# Autodesk Inventor assembly: LargeCaseAssembleV02
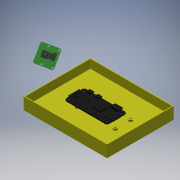
[picture p0: Inventor's stored thumbnail of the model, 180x180]
Saved by Autodesk Inventor 2019.4 (Build 234330000, 330)
## iProperties
Created: 2019-06-07
Part Number: LargeCaseAssembleV02
Document SubType Name: Assembly
Designer: steele
Author: steele
## Documents named in this file (4)
- C:\git\CAD-Development\robSteele\ShapeWays\TelescopeProjects\PiZeroWCamera\LargeCaseAssembleV02.iam
- C:\git\CAD-Development\robSteele\ShapeWays\TelescopeProjects\PiZeroWCamera\LargeCaseCaseBottomForPiZeroWV02.ipt
- C:\git\CAD-Development\robSteele\ShapeWays\TelescopeProjects\PiZeroWCamera\Pi_Zero_W_ThingIVerse.ipt
- C:\git\CAD-Development\robSteele\ShapeWays\TelescopeProjects\PiCameraThingiVerse\RPi_Camera_Module_v2.iam
## Components (3 placed, 3 different names)
1. LargeCaseCaseBottomForPiZeroWV02:1 — Mate:1, Mate:2, Mate:3
2. Pi_Zero_W_ThingIVerse:1 — Mate:1, Mate:2, Mate:3
3. RPi_Camera_Module_v2:1 [sub-assembly]
## Relationships (3: Mate 3)
- Mate:1: LargeCaseCaseBottomForPiZeroWV02:1 ↔ Pi_Zero_W_ThingIVerse:1
- Mate:2: LargeCaseCaseBottomForPiZeroWV02:1 ↔ Pi_Zero_W_ThingIVerse:1
- Mate:3: LargeCaseCaseBottomForPiZeroWV02:1 ↔ Pi_Zero_W_ThingIVerse:1
